# Autodesk Inventor assembly: MecanumWheel3.0
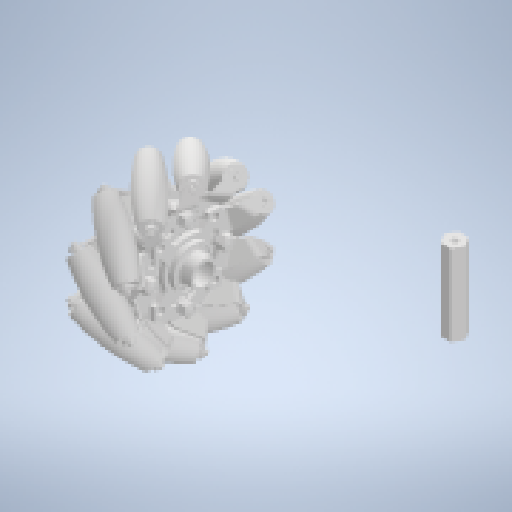
[picture p0: Inventor's stored thumbnail of the model, 512x512]
Saved by Autodesk Inventor 2023 (Build 270158000, 158)
## iProperties
Created: 2022-09-23
Part Number: MecanumWheel3.0
Document SubType Name: Assembly
Designer: deli
Author: deli
## Documents named in this file (7)
- C:\Users\deli\OneDrive - Eastside Preparatory School\FTC\8103-power-play\CAD\MecanumWheel3.0.iam
- C:\Users\deli\OneDrive - Eastside Preparatory School\FTC\8103-power-play\CAD\FTC-parts\goBILDA\3213-3606-0002\3606-0000-0096 assembly.ipt
- C:\Users\deli\OneDrive - Eastside Preparatory School\FTC\8103-power-play\CAD\FTC-parts\goBILDA\1603-0032-0012 assembly.ipt
- C:\Users\deli\OneDrive - Eastside Preparatory School\FTC\8103-power-play\CAD\6.5mmSpacer.ipt
- C:\Users\deli\OneDrive - Eastside Preparatory School\FTC\8103-power-play\CAD\wheelBearingInside3.0.ipt
- C:\Users\deli\OneDrive - Eastside Preparatory School\FTC\8103-power-play\CAD\17.5mmSpacer.ipt
- C:\Users\deli\OneDrive - Eastside Preparatory School\FTC\8103-power-play\CAD\FTC-parts\goBILDA\2104-0012-0048.ipt
## Components (7 placed, 6 different names)
1. 3606-0000-0096 assembly:1 — Mate:1, Mate:2, Mate:3, Mate:4, Mate:5, Mate:6
2. 1603-0032-0012 assembly:1 — Mate:1, Mate:2, Mate:3, Mate:13, Mate:14
3. 1603-0032-0012 assembly:2 — Mate:4, Mate:5, Mate:6, Mate:15, Mate:16, Mate:17, Mate:18, Mate:19
4. 6.5mmSpacer:1 — Mate:13, Mate:14, Flush:1, Mate:20
5. wheelBearingInside3.0:1 — Mate:15, Mate:16, Mate:17
6. 17.5mmSpacer:1 — Mate:18, Mate:19
7. 2104-0012-0048:1 — Flush:1, Mate:20
## Relationships (15: Mate 14, Flush 1)
- Mate:1: 3606-0000-0096 assembly:1 ↔ 1603-0032-0012 assembly:1
- Mate:2: 3606-0000-0096 assembly:1 ↔ 1603-0032-0012 assembly:1
- Mate:3: 3606-0000-0096 assembly:1 ↔ 1603-0032-0012 assembly:1
- Mate:4: 3606-0000-0096 assembly:1 ↔ 1603-0032-0012 assembly:2
- Mate:5: 3606-0000-0096 assembly:1 ↔ 1603-0032-0012 assembly:2
- Mate:6: 3606-0000-0096 assembly:1 ↔ 1603-0032-0012 assembly:2
- Mate:13: 1603-0032-0012 assembly:1 ↔ 6.5mmSpacer:1
- Mate:14: 1603-0032-0012 assembly:1 ↔ 6.5mmSpacer:1
- Mate:15: 1603-0032-0012 assembly:2 ↔ wheelBearingInside3.0:1
- Mate:16: 1603-0032-0012 assembly:2 ↔ wheelBearingInside3.0:1
- Mate:17: 1603-0032-0012 assembly:2 ↔ wheelBearingInside3.0:1
- Mate:18: 1603-0032-0012 assembly:2 ↔ 17.5mmSpacer:1
- Mate:19: 1603-0032-0012 assembly:2 ↔ 17.5mmSpacer:1
- Flush:1: 6.5mmSpacer:1 ↔ 2104-0012-0048:1
- Mate:20: 6.5mmSpacer:1 ↔ 2104-0012-0048:1
